# Autodesk Inventor assembly: omni wheel to hex shaft
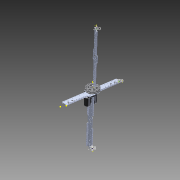
[picture p0: Inventor's stored thumbnail of the model, 180x180]
Saved by Autodesk Inventor 2015 (Build 190159000, 159)
## iProperties
Created: 2015-01-14
Part Number: omni wheel to hex shaft
Document SubType Name: Assembly
Designer: Robert
Author: Robert
## Documents named in this file (5)
- C:\Users\jhirshland1\Inventor\HWRobot2015\omni wheel to hex shaft.iam
- C:\Users\jhirshland1\Inventor\HWRobot2015\FRCKOP2015\AndyMark\217-2585.20121203.iam
- C:\Users\jhirshland1\Inventor\HWRobot2015\FRCKOP2015\AndyMark\am-2952+AM14U2+Inside+Sheet.ipt
- C:\Users\jhirshland1\Inventor\HWRobot2015\FRCKOP2015\Drive Base\Toughbox Mini L-Base.iam
- C:\Users\jhirshland1\Inventor\HWRobot2015\FRCKOP2015\Drive Base\FR8ZZ Hex Bearing.ipt
## Components (6 placed, 4 different names)
1. 217-2585.20121203:1 [sub-assembly] — Insert:1, Insert:2, Insert:3, Insert:4
2. am-2952+AM14U2+Inside+Sheet:1 — Insert:1, Insert:2, Mate:1, Mate:2
3. am-2952+AM14U2+Inside+Sheet:2 — Insert:3, Insert:4
4. Toughbox Mini L-Base:1 [sub-assembly] — Mate:1, Mate:2, Mate:3, Mate:4, Insert:5, Insert:6
5. FR8ZZ Hex Bearing:1 — Mate:3, Mate:4
6. am-2952+AM14U2+Inside+Sheet:1 — Insert:5, Insert:6
## Relationships (10: Insert 6, Mate 4)
- Insert:1: 217-2585.20121203:1 ↔ am-2952+AM14U2+Inside+Sheet:1
- Insert:2: 217-2585.20121203:1 ↔ am-2952+AM14U2+Inside+Sheet:1
- Insert:3: 217-2585.20121203:1 ↔ am-2952+AM14U2+Inside+Sheet:2
- Insert:4: 217-2585.20121203:1 ↔ am-2952+AM14U2+Inside+Sheet:2
- Mate:1: am-2952+AM14U2+Inside+Sheet:1 ↔ Toughbox Mini L-Base:1
- Mate:2: am-2952+AM14U2+Inside+Sheet:1 ↔ Toughbox Mini L-Base:1
- Mate:3: Toughbox Mini L-Base:1 ↔ FR8ZZ Hex Bearing:1
- Mate:4: Toughbox Mini L-Base:1 ↔ FR8ZZ Hex Bearing:1
- Insert:5: Toughbox Mini L-Base:1 ↔ am-2952+AM14U2+Inside+Sheet:1
- Insert:6: Toughbox Mini L-Base:1 ↔ am-2952+AM14U2+Inside+Sheet:1
